# Autodesk Inventor assembly: сборка серва 90
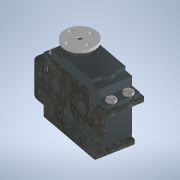
[picture p0: Inventor's stored thumbnail of the model, 180x180]
Saved by Autodesk Inventor 2020.1 (Build 241239000, 239)
## iProperties
Created: 2021-08-12
Part Number: сборка серва 90
Document SubType Name: Assembly
Designer: User
Author: User
## Documents named in this file (6)
- D:\GitHub\avatar-kvantoriada\3D\сборка серва 90.iam
- D:\GitHub\avatar-kvantoriada\3D\Деталь4.ipt
- D:\GitHub\avatar-kvantoriada\3D\MG996R.ipt
- D:\GitHub\avatar-kvantoriada\3D\Деталь5.ipt
- C:\Users\User\Documents\Inventor\Content Center Files\R2020\ru-RU\AS 1474(1)\AS 1474 - M3(1).ipt
- C:\Users\User\Documents\Inventor\Content Center Files\R2020\ru-RU\AS 1427(08)\AS 1427 - M3 x 8(6) I.ipt
## Components (11 placed, 5 different names)
1. Деталь4:1 — Жесткий:1, Жесткий:6, Жесткий:7, Жесткий:8, Жесткий:9
2. MG996R:1 — Жесткий:1, Совмещение:1, Совмещение:2, Жесткий:2, Жесткий:3, Жесткий:4, Жесткий:5
3. Деталь5:2 — Совмещение:1, Совмещение:2
4. AS 1427 Z - метрическая M3 x 8:6 — Жесткий:3
5. AS 1427 Z - метрическая M3 x 8:7 — Жесткий:2
6. AS 1427 Z - метрическая M3 x 8:8 — Жесткий:5
7. AS 1427 Z - метрическая M3 x 8:9 — Жесткий:4
8. AS 1474 - метрическая M3:2 — Жесткий:8
9. AS 1474 - метрическая M3:3 — Жесткий:7
10. AS 1474 - метрическая M3:4 — Жесткий:6
11. AS 1474 - метрическая M3:5 — Жесткий:9
## Relationships (11: WeldJoint 9, Mate 2)
- Жесткий:1 [WeldJoint]: Деталь4:1 ↔ MG996R:1
- Совмещение:1 [Mate]: MG996R:1 ↔ Деталь5:2
- Совмещение:2 [Mate]: MG996R:1 ↔ Деталь5:2
- Жесткий:2 [WeldJoint]: MG996R:1 ↔ AS 1427 Z - метрическая M3 x 8:7
- Жесткий:3 [WeldJoint]: MG996R:1 ↔ AS 1427 Z - метрическая M3 x 8:6
- Жесткий:4 [WeldJoint]: MG996R:1 ↔ AS 1427 Z - метрическая M3 x 8:9
- Жесткий:5 [WeldJoint]: MG996R:1 ↔ AS 1427 Z - метрическая M3 x 8:8
- Жесткий:6 [WeldJoint]: Деталь4:1 ↔ AS 1474 - метрическая M3:4
- Жесткий:7 [WeldJoint]: Деталь4:1 ↔ AS 1474 - метрическая M3:3
- Жесткий:8 [WeldJoint]: Деталь4:1 ↔ AS 1474 - метрическая M3:2
- Жесткий:9 [WeldJoint]: Деталь4:1 ↔ AS 1474 - метрическая M3:5
